# Autodesk Inventor assembly: Assembly1
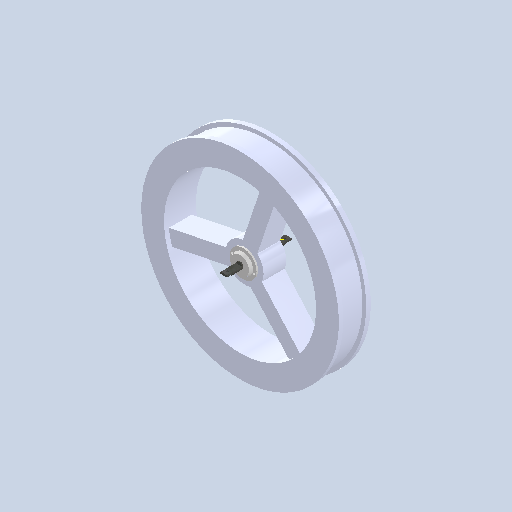
[picture p0: Inventor's stored thumbnail of the model, 512x512]
Saved by Autodesk Inventor 2025.2 (Build 292293000, 293)
## iProperties
Created: 2025-05-25
Part Number: Assembly1
Document SubType Name: Assembly
Designer: Moaz
Author: Moaz
## iProperties of the stored document PULLY.ipt
Created: 2025-05-24
Part Number: PULLY
Material: Generic
Document SubType Name: Modeling
Designer: Moaz
Density: 1 g/cm^3
Appearance: Default
Sending System: SolidWorks 2019
Last Author: Moaz
Last Saved: 2025-05-25
Author: Moaz
## Documents named in this file (8)
- D:\ASU\senior 1\semster 2\Advanced Manufacturing Technology & Prototyping\Project\Final Assembly\Project1\New folder (2)\Assembly1.iam
- D:\ASU\senior 1\semster 2\Advanced Manufacturing Technology & Prototyping\Project\Final Assembly\Project1\New folder (2)\Shaft.ipt
- D:\ASU\senior 1\semster 2\Advanced Manufacturing Technology & Prototyping\Project\Final Assembly\Project1\New folder (2)\SKF6213.ipt
- D:\ASU\senior 1\semster 2\Advanced Manufacturing Technology & Prototyping\Project\Final Assembly\Project1\New folder (2)\Cover.ipt
- D:\ASU\senior 1\semster 2\Advanced Manufacturing Technology & Prototyping\Project\Final Assembly\Project1\New folder (2)\DIN 555-5 - M48.ipt
- **D:\ASU\senior 1\semster 2\Advanced Manufacturing Technology & Prototyping\Project\Final Assembly\Project1\New folder (2)\Assembly1.iam*LocalDocs*xAaaaqabaAaaaaaaaAaaaqepv1b*PULLY.ipt
- **C:\Users\abdal\Desktop\P&Go\Assembly1.iam*LocalDocs*xAaaaqabaAaaaaaaaAaaaqepv1b*PULLY.ipt
- D:\ASU\senior 1\semster 2\Advanced Manufacturing Technology & Prototyping\Project\Final Assembly\Project1\New folder (2)\PULLY.SLDPRT
## Components (8 placed, 5 different names)
1. Shaft:1 — Mate:1, Mate:2, Mate:3, Mate:4, Mate:12, Mate:14, Mate:16, Mate:18, Mate:21
2. SKF- Single row ball bearings SKF6213:1 — Mate:1, Mate:3, Mate:15, Mate:17, Mate:20
3. SKF- Single row ball bearings SKF6213:2 — Mate:2, Mate:4, Mate:13, Mate:23
4. DIN 555 - replaced by DIN EN 24034 M48:1 — Mate:12, Mate:13
5. DIN 555 - replaced by DIN EN 24034 M48:2 — Mate:14, Mate:15
6. PULLY:1 — Mate:16, Mate:17, Mate:19, Mate:22
7. Cover:1 — Mate:18, Mate:19, Mate:20
8. Cover:2 — Mate:21, Mate:22, Mate:23
## Relationships (16: Mate 16)
- Mate:1: Shaft:1 ↔ SKF- Single row ball bearings SKF6213:1
- Mate:2: Shaft:1 ↔ SKF- Single row ball bearings SKF6213:2
- Mate:3: Shaft:1 ↔ SKF- Single row ball bearings SKF6213:1
- Mate:4: Shaft:1 ↔ SKF- Single row ball bearings SKF6213:2
- Mate:12: Shaft:1 ↔ DIN 555 - replaced by DIN EN 24034 M48:1
- Mate:13: SKF- Single row ball bearings SKF6213:2 ↔ DIN 555 - replaced by DIN EN 24034 M48:1
- Mate:14: Shaft:1 ↔ DIN 555 - replaced by DIN EN 24034 M48:2
- Mate:15: SKF- Single row ball bearings SKF6213:1 ↔ DIN 555 - replaced by DIN EN 24034 M48:2
- Mate:16: Shaft:1 ↔ PULLY:1
- Mate:17: SKF- Single row ball bearings SKF6213:1 ↔ PULLY:1
- Mate:18: Shaft:1 ↔ Cover:1
- Mate:19: PULLY:1 ↔ Cover:1
- Mate:20: SKF- Single row ball bearings SKF6213:1 ↔ Cover:1
- Mate:21: Shaft:1 ↔ Cover:2
- Mate:22: PULLY:1 ↔ Cover:2
- Mate:23: SKF- Single row ball bearings SKF6213:2 ↔ Cover:2
